# Autodesk Inventor assembly: Omnicscope_Xiao
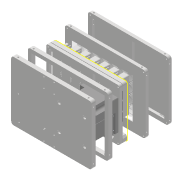
[picture p0: Inventor's stored thumbnail of the model, 180x180]
Saved by Autodesk Inventor 2022 (Build 260153000, 153)
## iProperties
Created: 2023-05-17
Part Number: Omnicscope_Xiao
Document SubType Name: Assembly
Designer: diederichbenedict
Author: diederichbenedict
## Documents named in this file (16)
- C:\Users\diederichbenedict\Dropbox\Dokumente\Promotion\PROJECTS\Omniscope\INVENTOR\Omnicscope_Xiao.iam
- C:\Users\diederichbenedict\Dropbox\Dokumente\Promotion\PROJECTS\Omniscope\INVENTOR\00_Omniscope_PCB_USBC.ipt
- C:\Users\diederichbenedict\Dropbox\Dokumente\Promotion\PROJECTS\Omniscope\INVENTOR\00_Seeeduino Xiao.ipt
- C:\Users\diederichbenedict\Dropbox\Dokumente\Promotion\PROJECTS\Omniscope\INVENTOR\Omniscope_USBC_Base_Top+.ipt
- C:\Users\diederichbenedict\Dropbox\Dokumente\Promotion\PROJECTS\Omniscope\INVENTOR\Omniscope_USBC_Bar.ipt
- C:\Users\diederichbenedict\Dropbox\Dokumente\Promotion\PROJECTS\Omniscope\INVENTOR\00_24wellplate_base.ipt
- C:\Users\diederichbenedict\Dropbox\Dokumente\Promotion\PROJECTS\Omniscope\INVENTOR\Omniscope_USBC_Wellplatemount.ipt
- C:\Users\diederichbenedict\Dropbox\Dokumente\Promotion\PROJECTS\Omniscope\INVENTOR\Omniscope_USBC_Base_Bottom.ipt
- C:\Users\diederichbenedict\Dropbox\Dokumente\Promotion\PROJECTS\Omniscope\INVENTOR\Omniscope_USBC_Bar_lenses.ipt
- C:\Users\diederichbenedict\Dropbox\Dokumente\Promotion\PROJECTS\Omniscope\INVENTOR\00_linear_z_stage_60mm.ipt
- C:\Users\diederichbenedict\Dropbox\Dokumente\Promotion\PROJECTS\Omniscope\INVENTOR\Omniscope_USBC_Base.ipt
- C:\Users\diederichbenedict\Dropbox\Dokumente\Promotion\PROJECTS\Omniscope\INVENTOR\Omniscope_USBC_Illuminationunit.ipt
- C:\Users\diederichbenedict\Dropbox\Dokumente\Promotion\PROJECTS\Omniscope\INVENTOR\Omniscope_USBC_Case.ipt
- C:\Users\diederichbenedict\Dropbox\Dokumente\Promotion\PROJECTS\Omniscope\INVENTOR\Omniscope_USBC_Wellplatemount2.ipt
- C:\Users\diederichbenedict\Dropbox\Dokumente\Promotion\PROJECTS\Omniscope\INVENTOR\Omniscope_USBC_labellid.ipt
- C:\Users\diederichbenedict\Dropbox\Dokumente\Promotion\PROJECTS\Omniscope\INVENTOR\00_Arduino_CNC_Assembly.ipt
## Components (48 placed, 15 different names)
1. 00_Omniscope_PCB_USBC:1 — Passend:1, Winkel:1, Passend:2, Passend:3, Fluchtend:1, Fluchtend:2, Fluchtend:8, Fluchtend:9
2. Omniscope_USBC_Base_Top+:1 — Fluchtend:1, Fluchtend:2, Fluchtend:3, Fluchtend:4
3. 00_24wellplate_base:1 — Fluchtend:5, Fluchtend:6, Fluchtend:7
4. Omniscope_USBC_Wellplatemount2:1 — Fluchtend:7
5. Omniscope_USBC_Base_Bottom:1 — Fluchtend:8, Fluchtend:9, Einfügen:1, Winkel:2
6. 00_linear_z_stage_60mm:1 — Einfügen:1, Winkel:2, Fluchtend:13, Fluchtend:14, Fluchtend:15
7. Omniscope_USBC_Base:1 — Fluchtend:13, Fluchtend:14, Fluchtend:15, Fluchtend:16, Fluchtend:17, Passend:4, Fluchtend:20, Fluchtend:21
8. Omniscope_USBC_Case:1 — Fluchtend:16, Fluchtend:17, Fluchtend:18, Fluchtend:19, Passend:5, Passend:6
9. Omniscope_USBC_Wellplatelifter:2
10. Omniscope_USBC_labellid:1 — Fluchtend:18, Fluchtend:19
11. 00_Arduino_CNC_Assembly:1 — Passend:4, Fluchtend:20, Fluchtend:21
12. Omniscope_USBC_Illuminationunit:2 — Passend:5, Passend:6
13. 00_Seeeduino Xiao:1 — Passend:1, Winkel:1, Passend:2, Passend:3
14. 00_Seeeduino Xiao:2
15. 00_Seeeduino Xiao:3
16. 00_Seeeduino Xiao:4
17. 00_Seeeduino Xiao:5
18. 00_Seeeduino Xiao:6 — Symmetrie:1
19. 00_Seeeduino Xiao:7
20. 00_Seeeduino Xiao:8
21. 00_Seeeduino Xiao:9
22. 00_Seeeduino Xiao:10
23. 00_Seeeduino Xiao:11
24. 00_Seeeduino Xiao:12
25. 00_Seeeduino Xiao:13
26. 00_Seeeduino Xiao:14
27. 00_Seeeduino Xiao:15 — Fluchtend:5
28. 00_Seeeduino Xiao:16
29. 00_Seeeduino Xiao:17
30. 00_Seeeduino Xiao:18
31. 00_Seeeduino Xiao:19 — Fluchtend:12
32. 00_Seeeduino Xiao:20
33. 00_Seeeduino Xiao:21
34. 00_Seeeduino Xiao:22 — Fluchtend:6
35. 00_Seeeduino Xiao:23 — Symmetrie:1
36. 00_Seeeduino Xiao:24
37. Omniscope_USBC_Bar:1 — Fluchtend:3, Fluchtend:4, Fluchtend:10, Fluchtend:11
38. Omniscope_USBC_Bar_lenses:1 — Fluchtend:10, Fluchtend:11, Fluchtend:12
39. Omniscope_USBC_Bar:2
40. Omniscope_USBC_Bar_lenses:2
41. Omniscope_USBC_Bar:3
42. Omniscope_USBC_Bar_lenses:3
43. Omniscope_USBC_Bar:4
44. Omniscope_USBC_Bar_lenses:4
45. Omniscope_USBC_Bar:5
46. Omniscope_USBC_Bar_lenses:5
47. Omniscope_USBC_Bar:6
48. Omniscope_USBC_Bar_lenses:6
## Component patterns: (24 elements, first: 00_Seeeduino Xiao:1), (6 elements, first: Omniscope_USBC_Bar:1 + Omniscope_USBC_Bar_lenses:1)
## Relationships (31: Flush 21, Mate 6, Angle 2, Symmetry 1, Insert 1)
- Passend:1 [Mate]: 00_Omniscope_PCB_USBC:1 ↔ 00_Seeeduino Xiao:1
- Winkel:1 [Angle] (0 deg): 00_Omniscope_PCB_USBC:1 ↔ 00_Seeeduino Xiao:1
- Passend:2 [Mate]: 00_Omniscope_PCB_USBC:1 ↔ 00_Seeeduino Xiao:1
- Passend:3 [Mate] (2 mm): 00_Omniscope_PCB_USBC:1 ↔ 00_Seeeduino Xiao:1
- Fluchtend:1 [Flush]: 00_Omniscope_PCB_USBC:1 ↔ Omniscope_USBC_Base_Top+:1
- Fluchtend:2 [Flush]: 00_Omniscope_PCB_USBC:1 ↔ Omniscope_USBC_Base_Top+:1
- Fluchtend:3 [Flush]: Omniscope_USBC_Base_Top+:1 ↔ Omniscope_USBC_Bar:1
- Fluchtend:4 [Flush]: Omniscope_USBC_Base_Top+:1 ↔ Omniscope_USBC_Bar:1
- Symmetrie:1: 00_Seeeduino Xiao:6 ↔ 00_Seeeduino Xiao:23
- Fluchtend:5 [Flush] (-0.5 mm): 00_24wellplate_base:1 ↔ 00_Seeeduino Xiao:15
- Fluchtend:6 [Flush] (-2 mm): 00_24wellplate_base:1 ↔ 00_Seeeduino Xiao:22
- Fluchtend:7 [Flush]: 00_24wellplate_base:1 ↔ Omniscope_USBC_Wellplatemount2:1
- Fluchtend:8 [Flush]: 00_Omniscope_PCB_USBC:1 ↔ Omniscope_USBC_Base_Bottom:1
- Fluchtend:9 [Flush]: 00_Omniscope_PCB_USBC:1 ↔ Omniscope_USBC_Base_Bottom:1
- Fluchtend:10 [Flush]: Omniscope_USBC_Bar:1 ↔ Omniscope_USBC_Bar_lenses:1
- Fluchtend:11 [Flush]: Omniscope_USBC_Bar:1 ↔ Omniscope_USBC_Bar_lenses:1
- Fluchtend:12 [Flush]: 00_Seeeduino Xiao:19 ↔ Omniscope_USBC_Bar_lenses:1
- Einfügen:1 [Insert]: Omniscope_USBC_Base_Bottom:1 ↔ 00_linear_z_stage_60mm:1
- Winkel:2 [Angle] (0 deg): Omniscope_USBC_Base_Bottom:1 ↔ 00_linear_z_stage_60mm:1
- Fluchtend:13 [Flush]: 00_linear_z_stage_60mm:1 ↔ Omniscope_USBC_Base:1
- Fluchtend:14 [Flush]: 00_linear_z_stage_60mm:1 ↔ Omniscope_USBC_Base:1
- Fluchtend:15 [Flush]: 00_linear_z_stage_60mm:1 ↔ Omniscope_USBC_Base:1
- Fluchtend:16 [Flush]: Omniscope_USBC_Base:1 ↔ Omniscope_USBC_Case:1
- Fluchtend:17 [Flush]: Omniscope_USBC_Base:1 ↔ Omniscope_USBC_Case:1
- Fluchtend:18 [Flush]: Omniscope_USBC_Case:1 ↔ Omniscope_USBC_labellid:1
- Fluchtend:19 [Flush]: Omniscope_USBC_Case:1 ↔ Omniscope_USBC_labellid:1
- Passend:4 [Mate] (1 mm): Omniscope_USBC_Base:1 ↔ 00_Arduino_CNC_Assembly:1
- Fluchtend:20 [Flush]: Omniscope_USBC_Base:1 ↔ 00_Arduino_CNC_Assembly:1
- Fluchtend:21 [Flush] (8 mm): Omniscope_USBC_Base:1 ↔ 00_Arduino_CNC_Assembly:1
- Passend:5 [Mate]: Omniscope_USBC_Case:1 ↔ Omniscope_USBC_Illuminationunit:2
- Passend:6 [Mate]: Omniscope_USBC_Case:1 ↔ Omniscope_USBC_Illuminationunit:2
